# Autodesk Inventor assembly: ParallelMechanismus_Driven_Assembly_v2.1_Rillenkugellager_Anlaufscheibe
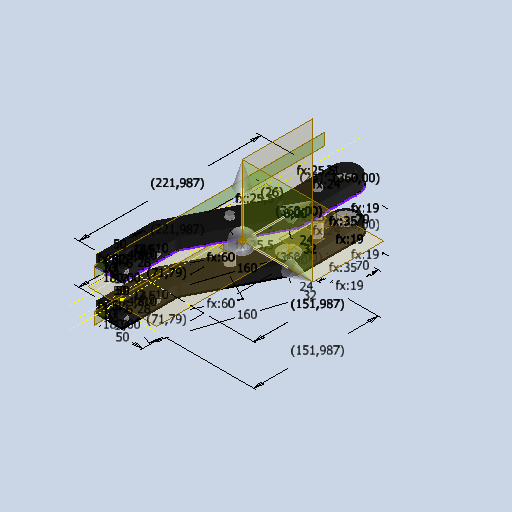
[picture p0: Inventor's stored thumbnail of the model, 512x512]
Saved by Autodesk Inventor 2024 (Build 280153000, 153)
## iProperties
Created: 2022-07-21
Part Number: ParallelMechanismus_Driven_Assembly_v2.1_Rillenkugellager_Anlaufscheibe
Document SubType Name: Assembly
Designer: alexw
Mass: 430.705 g
Surface Area: 757.391 cm^2
Volume: 208.944 cm^3
ParallelMecha_Contact_Dist: 26,000 mm
d167: 26,000 mm
d187: 26,000 mm
Author: alexw
## Documents named in this file (12)
- C:\Users\AEWALDER\Documents\Inventor\03_CurrentProjects\MasterThesis\PSM_V1_Rillenkugellager\ParallelMechanismus_Driven_Assembly_v2.1_Rillenkugellager_Anlaufscheibe.iam
- C:\Users\AEWALDER\Documents\Inventor\03_CurrentProjects\MasterThesis\PSM_V1_Rillenkugellager\ISO 7090 - 5 - 140 HV(1).ipt
- C:\Users\AEWALDER\Documents\Inventor\03_CurrentProjects\MasterThesis\PSM_V1_Rillenkugellager\ISO 4017 - M5 x 10 - ISO.ipt
- C:\Users\AEWALDER\Documents\Inventor\03_CurrentProjects\MasterThesis\PSM_V1_Rillenkugellager\ParallelSystem_ProximalPart_Driven_v2.1_Rillenkugellager.ipt
- C:\Users\AEWALDER\Documents\Inventor\03_CurrentProjects\MasterThesis\PSM_V1_Rillenkugellager\ParallelSystem_ProximalPart_Querstreben_v2_Rillenkugellager.ipt
- C:\Users\AEWALDER\Documents\Inventor\03_CurrentProjects\MasterThesis\PSM_V1_Rillenkugellager\SKF_W 61800 R-2RS1.iam
- C:\Users\AEWALDER\Documents\Inventor\03_CurrentProjects\MasterThesis\PSM_V1_Rillenkugellager\SKF_PCMW 122401_5 E.ipt
- C:\Users\AEWALDER\Documents\Inventor\03_CurrentProjects\MasterThesis\PSM_V1_Rillenkugellager\SKF_W 61800 R-2RS1_MIR.iam
- C:\Users\AEWALDER\Documents\Inventor\03_CurrentProjects\MasterThesis\PSM_V1_Rillenkugellager\SKF_PCMW 122401_5 E_MIR.ipt
- C:\Users\AEWALDER\Documents\Inventor\03_CurrentProjects\MasterThesis\PSM_V1_Rillenkugellager\ContentCenter\de-DE\ISO 4762(2)\ISO 4762 - M4 x 25ISO.ipt
- C:\Users\AEWALDER\Documents\Inventor\03_CurrentProjects\MasterThesis\PSM_V1_Rillenkugellager\ParallelSystem_ProximalPart_Driven_v2.1_Rillenkugellager_MIR1.ipt
- C:\Users\AEWALDER\Documents\Inventor\03_CurrentProjects\MasterThesis\PSM_V1_Rillenkugellager\ParallelSystem_ProximalPart_Driven_Counterpart.ipt
## Components (26 placed, 11 different names)
1. ParallelSystem_ProximalPart_Driven_v2.1_Rillenkugellager:1 — Fluchtend:1, Fluchtend:2, Fluchtend:3, Passend:62, Passend:63, Passend:64, Passend:65, Passend:67, Passend:68, Passend:69, Passend:72, Passend:78, Passend:79, Passend:80, Passend:81, Passend:91, Passend:92, Passend:116, Passend:117, Passend:132
2. ParallelSystem_ProximalPart_Querstreben_v2_Rillenkugellager:1 — Passend:48, Passend:50, Passend:56, Passend:58, Passend:62, Passend:63
3. ParallelSystem_ProximalPart_Querstreben_v2_Rillenkugellager:2 — Passend:46, Passend:52, Passend:54, Passend:60, Passend:64, Passend:65
4. ISO 7090 5 - 140 HV:1 — Passend:46, Passend:61, Passend:91
5. ISO 7090 5 - 140 HV:2 — Passend:48, Passend:59, Passend:92
6. ISO 7090 5 - 140 HV:3 — Passend:50, Passend:57, Passend:115
7. ISO 7090 5 - 140 HV:4 — Passend:52, Passend:55, Passend:114
8. ISO 4017 M5 x 10:1 — Passend:54, Passend:55
9. ISO 4017 M5 x 10:2 — Passend:56, Passend:57
10. ISO 4017 M5 x 10:3 — Passend:58, Passend:59
11. ISO 4017 M5 x 10:4 — Passend:60, Passend:61
12. SKF_W 61800 R-2RS1:4 [sub-assembly] — Passend:69, Passend:72
13. SKF_W 61800 R-2RS1:5 [sub-assembly] — Passend:67, Passend:68
14. SKF_PCMW 122401_5 E:2 — Passend:78, Passend:79
15. SKF_PCMW 122401_5 E:3 — Passend:80, Passend:81
16. SKF_W 61800 R-2RS1_MIR:1 [sub-assembly] — Passend:108, Passend:109, Passend:112, Passend:113
17. SKF_W 61800 R-2RS1_MIR:2 [sub-assembly] — Passend:106, Passend:107, Passend:110, Passend:111
18. SKF_PCMW 122401_5 E_MIR:1 — Passend:108, Passend:109
19. SKF_PCMW 122401_5 E_MIR:2 — Passend:106, Passend:107
20. ISO 4762 M4 x 25:1 — Passend:121, Passend:122
21. ISO 4762 M4 x 25:2 — Passend:126, Passend:127
22. ParallelSystem_ProximalPart_Driven_v2.1_Rillenkugellager_MIR1:1 — Passend:99, Fluchtend:6, Fluchtend:7, Passend:110, Passend:111, Passend:112, Passend:113, Passend:114, Passend:115, Passend:123, Passend:124, Passend:126, Passend:131
23. ISO 4762 M4 x 25:3 — Passend:119, Passend:120
24. ISO 4762 M4 x 25:4 — Passend:128, Passend:129
25. ParallelSystem_ProximalPart_Driven_Counterpart:1 — Passend:116, Passend:117, Passend:119, Passend:120, Passend:121, Passend:122, Passend:132
26. ParallelSystem_ProximalPart_Driven_Counterpart:2 — Passend:123, Passend:124, Passend:127, Passend:128, Passend:129, Passend:131
## Relationships (56: Mate 51, Flush 5)
- Fluchtend:1 [Flush]: ParallelSystem_ProximalPart_Driven_v2.1_Rillenkugellager:1
- Fluchtend:2 [Flush]: ParallelSystem_ProximalPart_Driven_v2.1_Rillenkugellager:1
- Fluchtend:3 [Flush]: ParallelSystem_ProximalPart_Driven_v2.1_Rillenkugellager:1
- Passend:46 [Mate]: ParallelSystem_ProximalPart_Querstreben_v2_Rillenkugellager:2 ↔ ISO 7090 5 - 140 HV:1
- Passend:48 [Mate]: ParallelSystem_ProximalPart_Querstreben_v2_Rillenkugellager:1 ↔ ISO 7090 5 - 140 HV:2
- Passend:50 [Mate]: ParallelSystem_ProximalPart_Querstreben_v2_Rillenkugellager:1 ↔ ISO 7090 5 - 140 HV:3
- Passend:52 [Mate]: ParallelSystem_ProximalPart_Querstreben_v2_Rillenkugellager:2 ↔ ISO 7090 5 - 140 HV:4
- Passend:54 [Mate]: ParallelSystem_ProximalPart_Querstreben_v2_Rillenkugellager:2 ↔ ISO 4017 M5 x 10:1
- Passend:55 [Mate]: ISO 7090 5 - 140 HV:4 ↔ ISO 4017 M5 x 10:1
- Passend:56 [Mate]: ParallelSystem_ProximalPart_Querstreben_v2_Rillenkugellager:1 ↔ ISO 4017 M5 x 10:2
- Passend:57 [Mate]: ISO 7090 5 - 140 HV:3 ↔ ISO 4017 M5 x 10:2
- Passend:58 [Mate]: ParallelSystem_ProximalPart_Querstreben_v2_Rillenkugellager:1 ↔ ISO 4017 M5 x 10:3
- Passend:59 [Mate]: ISO 7090 5 - 140 HV:2 ↔ ISO 4017 M5 x 10:3
- Passend:60 [Mate]: ParallelSystem_ProximalPart_Querstreben_v2_Rillenkugellager:2 ↔ ISO 4017 M5 x 10:4
- Passend:61 [Mate]: ISO 7090 5 - 140 HV:1 ↔ ISO 4017 M5 x 10:4
- Passend:62 [Mate]: ParallelSystem_ProximalPart_Driven_v2.1_Rillenkugellager:1 ↔ ParallelSystem_ProximalPart_Querstreben_v2_Rillenkugellager:1
- Passend:63 [Mate]: ParallelSystem_ProximalPart_Driven_v2.1_Rillenkugellager:1 ↔ ParallelSystem_ProximalPart_Querstreben_v2_Rillenkugellager:1
- Passend:64 [Mate]: ParallelSystem_ProximalPart_Driven_v2.1_Rillenkugellager:1 ↔ ParallelSystem_ProximalPart_Querstreben_v2_Rillenkugellager:2
- Passend:65 [Mate]: ParallelSystem_ProximalPart_Driven_v2.1_Rillenkugellager:1 ↔ ParallelSystem_ProximalPart_Querstreben_v2_Rillenkugellager:2
- Passend:67 [Mate]: ParallelSystem_ProximalPart_Driven_v2.1_Rillenkugellager:1 ↔ SKF_W 61800 R-2RS1:5
- Passend:68 [Mate]: ParallelSystem_ProximalPart_Driven_v2.1_Rillenkugellager:1 ↔ SKF_W 61800 R-2RS1:5
- Passend:69 [Mate]: ParallelSystem_ProximalPart_Driven_v2.1_Rillenkugellager:1 ↔ SKF_W 61800 R-2RS1:4
- Passend:72 [Mate]: ParallelSystem_ProximalPart_Driven_v2.1_Rillenkugellager:1 ↔ SKF_W 61800 R-2RS1:4
- Passend:78 [Mate]: ParallelSystem_ProximalPart_Driven_v2.1_Rillenkugellager:1 ↔ SKF_PCMW 122401_5 E:2
- Passend:79 [Mate]: ParallelSystem_ProximalPart_Driven_v2.1_Rillenkugellager:1 ↔ SKF_PCMW 122401_5 E:2
- Passend:80 [Mate]: ParallelSystem_ProximalPart_Driven_v2.1_Rillenkugellager:1 ↔ SKF_PCMW 122401_5 E:3
- Passend:81 [Mate]: ParallelSystem_ProximalPart_Driven_v2.1_Rillenkugellager:1 ↔ SKF_PCMW 122401_5 E:3
- Passend:91 [Mate]: ParallelSystem_ProximalPart_Driven_v2.1_Rillenkugellager:1 ↔ ISO 7090 5 - 140 HV:1
- Passend:92 [Mate]: ParallelSystem_ProximalPart_Driven_v2.1_Rillenkugellager:1 ↔ ISO 7090 5 - 140 HV:2
- Passend:99 [Mate]: ParallelSystem_ProximalPart_Driven_v2.1_Rillenkugellager_MIR1:1
- Fluchtend:6 [Flush]: ParallelSystem_ProximalPart_Driven_v2.1_Rillenkugellager_MIR1:1
- Fluchtend:7 [Flush]: ParallelSystem_ProximalPart_Driven_v2.1_Rillenkugellager_MIR1:1
- Passend:106 [Mate]: SKF_W 61800 R-2RS1_MIR:2 ↔ SKF_PCMW 122401_5 E_MIR:2
- Passend:107 [Mate]: SKF_W 61800 R-2RS1_MIR:2 ↔ SKF_PCMW 122401_5 E_MIR:2
- Passend:108 [Mate]: SKF_W 61800 R-2RS1_MIR:1 ↔ SKF_PCMW 122401_5 E_MIR:1
- Passend:109 [Mate]: SKF_W 61800 R-2RS1_MIR:1 ↔ SKF_PCMW 122401_5 E_MIR:1
- Passend:110 [Mate]: SKF_W 61800 R-2RS1_MIR:2 ↔ ParallelSystem_ProximalPart_Driven_v2.1_Rillenkugellager_MIR1:1
- Passend:111 [Mate]: SKF_W 61800 R-2RS1_MIR:2 ↔ ParallelSystem_ProximalPart_Driven_v2.1_Rillenkugellager_MIR1:1
- Passend:112 [Mate]: SKF_W 61800 R-2RS1_MIR:1 ↔ ParallelSystem_ProximalPart_Driven_v2.1_Rillenkugellager_MIR1:1
- Passend:113 [Mate]: SKF_W 61800 R-2RS1_MIR:1 ↔ ParallelSystem_ProximalPart_Driven_v2.1_Rillenkugellager_MIR1:1
- Passend:114 [Mate]: ISO 7090 5 - 140 HV:4 ↔ ParallelSystem_ProximalPart_Driven_v2.1_Rillenkugellager_MIR1:1
- Passend:115 [Mate]: ISO 7090 5 - 140 HV:3 ↔ ParallelSystem_ProximalPart_Driven_v2.1_Rillenkugellager_MIR1:1
- Passend:116 [Mate]: ParallelSystem_ProximalPart_Driven_v2.1_Rillenkugellager:1 ↔ ParallelSystem_ProximalPart_Driven_Counterpart:1
- Passend:117 [Mate]: ParallelSystem_ProximalPart_Driven_v2.1_Rillenkugellager:1 ↔ ParallelSystem_ProximalPart_Driven_Counterpart:1
- Passend:119 [Mate]: ISO 4762 M4 x 25:3 ↔ ParallelSystem_ProximalPart_Driven_Counterpart:1
- Passend:120 [Mate]: ISO 4762 M4 x 25:3 ↔ ParallelSystem_ProximalPart_Driven_Counterpart:1
- Passend:121 [Mate]: ISO 4762 M4 x 25:1 ↔ ParallelSystem_ProximalPart_Driven_Counterpart:1
- Passend:122 [Mate]: ISO 4762 M4 x 25:1 ↔ ParallelSystem_ProximalPart_Driven_Counterpart:1
- Passend:123 [Mate]: ParallelSystem_ProximalPart_Driven_v2.1_Rillenkugellager_MIR1:1 ↔ ParallelSystem_ProximalPart_Driven_Counterpart:2
- Passend:124 [Mate]: ParallelSystem_ProximalPart_Driven_v2.1_Rillenkugellager_MIR1:1 ↔ ParallelSystem_ProximalPart_Driven_Counterpart:2
- Passend:126 [Mate]: ISO 4762 M4 x 25:2 ↔ ParallelSystem_ProximalPart_Driven_v2.1_Rillenkugellager_MIR1:1
- Passend:127 [Mate]: ISO 4762 M4 x 25:2 ↔ ParallelSystem_ProximalPart_Driven_Counterpart:2
- Passend:128 [Mate]: ISO 4762 M4 x 25:4 ↔ ParallelSystem_ProximalPart_Driven_Counterpart:2
- Passend:129 [Mate]: ISO 4762 M4 x 25:4 ↔ ParallelSystem_ProximalPart_Driven_Counterpart:2
- Passend:131 [Mate]: ParallelSystem_ProximalPart_Driven_v2.1_Rillenkugellager_MIR1:1 ↔ ParallelSystem_ProximalPart_Driven_Counterpart:2
- Passend:132 [Mate]: ParallelSystem_ProximalPart_Driven_v2.1_Rillenkugellager:1 ↔ ParallelSystem_ProximalPart_Driven_Counterpart:1
## Named parameters: ParallelMecha_Contact_Dist = 26 mm
